# Autodesk Inventor assembly: M - Carriage
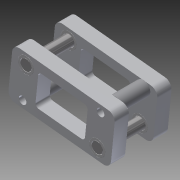
[picture p0: Inventor's stored thumbnail of the model, 180x180]
Saved by Autodesk Inventor 2013 (Build 170138000, 138)
## iProperties
Created: 2013-02-17
Part Number: M - Carriage
Document SubType Name: Assembly
Designer: Moses
Mass: 227.953 g
Surface Area: 382.736 cm^2
Volume: 73.7901 cm^3
Density: 3.0892 g/cm^3
Author: Moses
## Documents named in this file (5)
- C:\Users\Arpan\Documents\GitHub\frc2013CAD\M-Climber\M - Carriage.iam
- C:\Users\Arpan\Documents\GitHub\frc2013CAD\M-Climber\5905K220\5905K220.ipt
- C:\Users\Arpan\Documents\GitHub\frc2013CAD\M-Climber\M - 0.375 Shaft Carriage.ipt
- C:\Users\Arpan\Documents\GitHub\frc2013CAD\M-Climber\M - Carriage Plate Part 1.ipt
- C:\Users\Arpan\Documents\GitHub\frc2013CAD\M-Climber\M - 0.375 Aluminum Tube Spacer.ipt
## Components (10 placed, 4 different names)
1. M - 0.375 Shaft Carriage:1 — Mate:3, Mate:4, Flush:3
2. M - Carriage Plate Part 1:1 — Mate:3, Flush:2, Insert:1, Insert:3, Mate:5, Flush:3, Insert:5, Insert:6
3. M - Carriage Plate Part 1:2 — Mate:4, Flush:2, Insert:2, Insert:4, Mate:5, Insert:7
4. 5905K220:1 — Insert:2
5. 5905K220:2 — Insert:4
6. 5905K220:3 — Insert:1
7. 5905K220:4 — Insert:3
8. M - 0.375 Shaft Carriage:2 — Insert:5
9. M - 0.375 Aluminum Tube Spacer:1 — Insert:6
10. M - 0.375 Aluminum Tube Spacer:2 — Insert:7
## Relationships (12: Insert 7, Mate 3, Flush 2)
- Mate:3: M - 0.375 Shaft Carriage:1 ↔ M - Carriage Plate Part 1:1
- Mate:4: M - 0.375 Shaft Carriage:1 ↔ M - Carriage Plate Part 1:2
- Flush:2: M - Carriage Plate Part 1:1 ↔ M - Carriage Plate Part 1:2
- Insert:1: M - Carriage Plate Part 1:1 ↔ 5905K220:3
- Insert:2: M - Carriage Plate Part 1:2 ↔ 5905K220:1
- Insert:3: M - Carriage Plate Part 1:1 ↔ 5905K220:4
- Insert:4: M - Carriage Plate Part 1:2 ↔ 5905K220:2
- Mate:5 (25.4 mm): M - Carriage Plate Part 1:1 ↔ M - Carriage Plate Part 1:2
- Flush:3: M - 0.375 Shaft Carriage:1 ↔ M - Carriage Plate Part 1:1
- Insert:5: M - Carriage Plate Part 1:1 ↔ M - 0.375 Shaft Carriage:2
- Insert:6: M - Carriage Plate Part 1:1 ↔ M - 0.375 Aluminum Tube Spacer:1
- Insert:7: M - Carriage Plate Part 1:2 ↔ M - 0.375 Aluminum Tube Spacer:2
